# Autodesk Inventor assembly: Rack and Pinion Gearbox Assembly
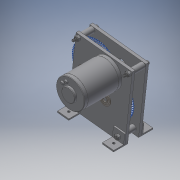
[picture p0: Inventor's stored thumbnail of the model, 180x180]
Saved by Autodesk Inventor 2018 (Build 220112000, 112)
## iProperties
Created: 2019-01-29
Part Number: Rack and Pinion Gearbox Assembly
Document SubType Name: Assembly
Designer: maste
Author: maste
## Documents named in this file (14)
- C:\Users\maste\OneDrive\Documents\GitHub\2019CAD\Drivebase but Calvin is a mad man\Rack and Pinion Gearbox Assembly.iam
- C:\Users\maste\OneDrive\Documents\GitHub\2019CAD\Drivebase but Calvin is a mad man\Rack and Pinion Gearbox Plate.ipt
- C:\Users\maste\OneDrive\Documents\GitHub\2019CAD\Drivebase but Calvin is a mad man\12t_Steel_Spur_Gear_20_DP_CIM_Motor_217-3099.ipt
- C:\Users\maste\OneDrive\Documents\GitHub\2019CAD\Drivebase but Calvin is a mad man\14t_Steel_Spur_Gear_20_DP_3_8_Hex_Bore_217-3100.step.ipt
- C:\Users\maste\OneDrive\Documents\GitHub\2019CAD\Drivebase but Calvin is a mad man\72t_Aluminum_Spur_Gear_20_DP_1_2_Hex_Bore_217-3576.ipt
- C:\Users\maste\OneDrive\Documents\GitHub\2019CAD\Drivebase but Calvin is a mad man\am-3832 375H to 500H Adapter.ipt
- C:\Users\maste\OneDrive\Documents\GitHub\2019CAD\Drivebase but Calvin is a mad man\Mini_CIM_Motor_217-3371.ipt
- C:\Users\maste\OneDrive\Documents\GitHub\2019CAD\Drivebase but Calvin is a mad man\10_25mm_3_8_ThunderHex_ID_x_0_875_OD_x_0_280_WD_Flanged_Bearing_217-5829 (1).ipt
- C:\Users\maste\OneDrive\Documents\GitHub\2019CAD\Drivebase but Calvin is a mad man\92196A272_18-8 STAINLESS STEEL SOCKET HEAD CAP SCREW.ipt
- C:\Users\maste\OneDrive\Documents\GitHub\2019CAD\Drivebase but Calvin is a mad man\Not Tiberculosis TB Hex Shaft.ipt
- C:\Users\maste\OneDrive\Documents\GitHub\2019CAD\Drivebase but Calvin is a mad man\I'm not awake enough to be making churros.ipt
- C:\Users\maste\OneDrive\Documents\GitHub\2019CAD\Drivebase but Calvin is a mad man\L-Bracket L.ipt
- C:\Users\maste\OneDrive\Documents\GitHub\2019CAD\Drivebase but Calvin is a mad man\92196A253_18-8 STAINLESS STEEL SOCKET HEAD CAP SCREW.ipt
- C:\Users\maste\OneDrive\Documents\GitHub\2019CAD\Drivebase but Calvin is a mad man\91831A011_TYPE 18-8 STAINLESS STL NYLON-INSERT LOCKNUT.ipt
## Components (33 placed, 13 different names)
1. Rack and Pinion Gearbox Plate:1 — Mate:79, Mate:80, Mate:81, Mate:82, Mate:94, Mate:95, Mate:97, Mate:98, Mate:99, Flush:4, Mate:101, Mate:102, Mate:103, Mate:105, Mate:106, Mate:107, Flush:5, Mate:109, Flush:6, Flush:7
2. Rack and Pinion Gearbox Plate:2 — Mate:68, Mate:69, Mate:70, Mate:71, Mate:72, Mate:73, Mate:74, Mate:75, Mate:76, Mate:77, Mate:78, Flush:6, Flush:7, Mate:110, Mate:111, Mate:112, Mate:113, Flush:8, Flush:9, Flush:10, Flush:11, Mate:114, Rotation:2, Rotation:3
3. 12t_Steel_Spur_Gear_20_DP_CIM_Motor_217-3099:1 — Mate:85, Flush:2, Mate:86
4. 14t_Steel_Spur_Gear_20_DP_3_8_Hex_Bore_217-3100.step:1 — Mate:21, Mate:22, Mate:92, Mate:93
5. 72t_Aluminum_Spur_Gear_20_DP_1_2_Hex_Bore_217-3576:1 — Mate:90, Mate:91, Flush:3
6. 72t_Aluminum_Spur_Gear_20_DP_1_2_Hex_Bore_217-3576:2 — Mate:83, Mate:84, Flush:1, Mate:89
7. am-3832 375H to 500H Adapter:1 — Mate:18, Mate:19, Mate:90, Mate:91, Flush:3, Mate:93
8. am-3832 375H to 500H Adapter:2 — Mate:32, Mate:33, Mate:83, Mate:84, Flush:1, Mate:87, Mate:88
9. Mini_CIM_Motor_217-3371:1 — Mate:68, Mate:69, Mate:70, Mate:85, Flush:2, Mate:86
10. 10_25mm_3_8_ThunderHex_ID_x_0_875_OD_x_0_280_WD_Flanged_Bearing_217-5829 (1):1 — Mate:73, Mate:74, Rotation:3
11. 10_25mm_3_8_ThunderHex_ID_x_0_875_OD_x_0_280_WD_Flanged_Bearing_217-5829 (1):2 — Mate:71, Mate:72, Rotation:1, Rotation:2
12. 10_25mm_3_8_ThunderHex_ID_x_0_875_OD_x_0_280_WD_Flanged_Bearing_217-5829 (1):3 — Mate:28, Mate:29, Mate:81, Mate:82, Mate:89
13. 10_25mm_3_8_ThunderHex_ID_x_0_875_OD_x_0_280_WD_Flanged_Bearing_217-5829 (1):4 — Mate:16, Mate:17, Mate:79, Mate:80, Mate:92
14. 92196A272_18-8 STAINLESS STEEL SOCKET HEAD CAP SCREW:1 — Mate:75, Mate:76
15. 92196A272_18-8 STAINLESS STEEL SOCKET HEAD CAP SCREW:2 — Mate:77, Mate:78
16. Not Tiberculosis TB Hex Shaft:1 — Mate:16, Mate:17, Mate:18, Mate:19, Mate:21, Mate:22, Rotation:1
17. Not Tiberculosis TB Hex Shaft:2 — Mate:28, Mate:29, Mate:32, Mate:33, Mate:87, Mate:88
18. I'm not awake enough to be making churros:1 — Mate:104, Mate:105
19. I'm not awake enough to be making churros:2 — Mate:96, Mate:97, Mate:110
20. I'm not awake enough to be making churros:3 — Mate:100, Mate:101
21. I'm not awake enough to be making churros:4 — Mate:108, Mate:109
22. L-Bracket L:1 — Mate:55, Mate:58, Mate:99, Flush:4
23. L-Bracket L:2 — Mate:54, Mate:59, Mate:107, Flush:5
24. L-Bracket L:3 — Mate:63, Flush:10, Flush:11, Mate:114
25. L-Bracket L:4 — Mate:62, Mate:113, Flush:8, Flush:9
26. 92196A253_18-8 STAINLESS STEEL SOCKET HEAD CAP SCREW:1 — Mate:54, Mate:59, Mate:65, Mate:106, Mate:108
27. 92196A253_18-8 STAINLESS STEEL SOCKET HEAD CAP SCREW:2 — Mate:55, Mate:58, Mate:64, Mate:98, Mate:100
28. 92196A253_18-8 STAINLESS STEEL SOCKET HEAD CAP SCREW:3 — Mate:67, Mate:94, Mate:95, Mate:96
29. 92196A253_18-8 STAINLESS STEEL SOCKET HEAD CAP SCREW:4 — Mate:66, Mate:102, Mate:103, Mate:104
30. 91831A011_TYPE 18-8 STAINLESS STL NYLON-INSERT LOCKNUT:1 — Mate:62, Mate:64
31. 91831A011_TYPE 18-8 STAINLESS STL NYLON-INSERT LOCKNUT:2 — Mate:63, Mate:65
32. 91831A011_TYPE 18-8 STAINLESS STL NYLON-INSERT LOCKNUT:3 — Mate:67, Mate:111
33. 91831A011_TYPE 18-8 STAINLESS STL NYLON-INSERT LOCKNUT:4 — Mate:66, Mate:112
## Relationships (81: Mate 67, Flush 11, RelateRotation 3)
- Mate:16: 10_25mm_3_8_ThunderHex_ID_x_0_875_OD_x_0_280_WD_Flanged_Bearing_217-5829 (1):4 ↔ Not Tiberculosis TB Hex Shaft:1
- Mate:17: 10_25mm_3_8_ThunderHex_ID_x_0_875_OD_x_0_280_WD_Flanged_Bearing_217-5829 (1):4 ↔ Not Tiberculosis TB Hex Shaft:1
- Mate:18: am-3832 375H to 500H Adapter:1 ↔ Not Tiberculosis TB Hex Shaft:1
- Mate:19: am-3832 375H to 500H Adapter:1 ↔ Not Tiberculosis TB Hex Shaft:1
- Mate:21: 14t_Steel_Spur_Gear_20_DP_3_8_Hex_Bore_217-3100.step:1 ↔ Not Tiberculosis TB Hex Shaft:1
- Mate:22: 14t_Steel_Spur_Gear_20_DP_3_8_Hex_Bore_217-3100.step:1 ↔ Not Tiberculosis TB Hex Shaft:1
- Mate:28: 10_25mm_3_8_ThunderHex_ID_x_0_875_OD_x_0_280_WD_Flanged_Bearing_217-5829 (1):3 ↔ Not Tiberculosis TB Hex Shaft:2
- Mate:29: 10_25mm_3_8_ThunderHex_ID_x_0_875_OD_x_0_280_WD_Flanged_Bearing_217-5829 (1):3 ↔ Not Tiberculosis TB Hex Shaft:2
- Mate:32: am-3832 375H to 500H Adapter:2 ↔ Not Tiberculosis TB Hex Shaft:2
- Mate:33: am-3832 375H to 500H Adapter:2 ↔ Not Tiberculosis TB Hex Shaft:2
- Mate:54: L-Bracket L:2 ↔ 92196A253_18-8 STAINLESS STEEL SOCKET HEAD CAP SCREW:1
- Mate:55: L-Bracket L:1 ↔ 92196A253_18-8 STAINLESS STEEL SOCKET HEAD CAP SCREW:2
- Mate:58: L-Bracket L:1 ↔ 92196A253_18-8 STAINLESS STEEL SOCKET HEAD CAP SCREW:2
- Mate:59: L-Bracket L:2 ↔ 92196A253_18-8 STAINLESS STEEL SOCKET HEAD CAP SCREW:1
- Mate:62: L-Bracket L:4 ↔ 91831A011_TYPE 18-8 STAINLESS STL NYLON-INSERT LOCKNUT:1
- Mate:63: L-Bracket L:3 ↔ 91831A011_TYPE 18-8 STAINLESS STL NYLON-INSERT LOCKNUT:2
- Mate:64: 92196A253_18-8 STAINLESS STEEL SOCKET HEAD CAP SCREW:2 ↔ 91831A011_TYPE 18-8 STAINLESS STL NYLON-INSERT LOCKNUT:1
- Mate:65: 92196A253_18-8 STAINLESS STEEL SOCKET HEAD CAP SCREW:1 ↔ 91831A011_TYPE 18-8 STAINLESS STL NYLON-INSERT LOCKNUT:2
- Mate:66: 92196A253_18-8 STAINLESS STEEL SOCKET HEAD CAP SCREW:4 ↔ 91831A011_TYPE 18-8 STAINLESS STL NYLON-INSERT LOCKNUT:4
- Mate:67: 92196A253_18-8 STAINLESS STEEL SOCKET HEAD CAP SCREW:3 ↔ 91831A011_TYPE 18-8 STAINLESS STL NYLON-INSERT LOCKNUT:3
- Mate:68: Rack and Pinion Gearbox Plate:2 ↔ Mini_CIM_Motor_217-3371:1
- Mate:69: Rack and Pinion Gearbox Plate:2 ↔ Mini_CIM_Motor_217-3371:1
- Mate:70: Rack and Pinion Gearbox Plate:2 ↔ Mini_CIM_Motor_217-3371:1
- Mate:71: Rack and Pinion Gearbox Plate:2 ↔ 10_25mm_3_8_ThunderHex_ID_x_0_875_OD_x_0_280_WD_Flanged_Bearing_217-5829 (1):2
- Mate:72: Rack and Pinion Gearbox Plate:2 ↔ 10_25mm_3_8_ThunderHex_ID_x_0_875_OD_x_0_280_WD_Flanged_Bearing_217-5829 (1):2
- Mate:73: Rack and Pinion Gearbox Plate:2 ↔ 10_25mm_3_8_ThunderHex_ID_x_0_875_OD_x_0_280_WD_Flanged_Bearing_217-5829 (1):1
- Mate:74: Rack and Pinion Gearbox Plate:2 ↔ 10_25mm_3_8_ThunderHex_ID_x_0_875_OD_x_0_280_WD_Flanged_Bearing_217-5829 (1):1
- Mate:75: Rack and Pinion Gearbox Plate:2 ↔ 92196A272_18-8 STAINLESS STEEL SOCKET HEAD CAP SCREW:1
- Mate:76: Rack and Pinion Gearbox Plate:2 ↔ 92196A272_18-8 STAINLESS STEEL SOCKET HEAD CAP SCREW:1
- Mate:77: Rack and Pinion Gearbox Plate:2 ↔ 92196A272_18-8 STAINLESS STEEL SOCKET HEAD CAP SCREW:2
- Mate:78: Rack and Pinion Gearbox Plate:2 ↔ 92196A272_18-8 STAINLESS STEEL SOCKET HEAD CAP SCREW:2
- Mate:79: Rack and Pinion Gearbox Plate:1 ↔ 10_25mm_3_8_ThunderHex_ID_x_0_875_OD_x_0_280_WD_Flanged_Bearing_217-5829 (1):4
- Mate:80: Rack and Pinion Gearbox Plate:1 ↔ 10_25mm_3_8_ThunderHex_ID_x_0_875_OD_x_0_280_WD_Flanged_Bearing_217-5829 (1):4
- Mate:81: Rack and Pinion Gearbox Plate:1 ↔ 10_25mm_3_8_ThunderHex_ID_x_0_875_OD_x_0_280_WD_Flanged_Bearing_217-5829 (1):3
- Mate:82: Rack and Pinion Gearbox Plate:1 ↔ 10_25mm_3_8_ThunderHex_ID_x_0_875_OD_x_0_280_WD_Flanged_Bearing_217-5829 (1):3
- Mate:83: 72t_Aluminum_Spur_Gear_20_DP_1_2_Hex_Bore_217-3576:2 ↔ am-3832 375H to 500H Adapter:2
- Mate:84: 72t_Aluminum_Spur_Gear_20_DP_1_2_Hex_Bore_217-3576:2 ↔ am-3832 375H to 500H Adapter:2
- Flush:1: 72t_Aluminum_Spur_Gear_20_DP_1_2_Hex_Bore_217-3576:2 ↔ am-3832 375H to 500H Adapter:2
- Mate:85: 12t_Steel_Spur_Gear_20_DP_CIM_Motor_217-3099:1 ↔ Mini_CIM_Motor_217-3371:1
- Flush:2: 12t_Steel_Spur_Gear_20_DP_CIM_Motor_217-3099:1 ↔ Mini_CIM_Motor_217-3371:1
- Mate:86: 12t_Steel_Spur_Gear_20_DP_CIM_Motor_217-3099:1 ↔ Mini_CIM_Motor_217-3371:1
- Mate:87: am-3832 375H to 500H Adapter:2 ↔ Not Tiberculosis TB Hex Shaft:2
- Mate:88: am-3832 375H to 500H Adapter:2 ↔ Not Tiberculosis TB Hex Shaft:2
- Mate:89: 72t_Aluminum_Spur_Gear_20_DP_1_2_Hex_Bore_217-3576:2 ↔ 10_25mm_3_8_ThunderHex_ID_x_0_875_OD_x_0_280_WD_Flanged_Bearing_217-5829 (1):3
- Mate:90: 72t_Aluminum_Spur_Gear_20_DP_1_2_Hex_Bore_217-3576:1 ↔ am-3832 375H to 500H Adapter:1
- Mate:91: 72t_Aluminum_Spur_Gear_20_DP_1_2_Hex_Bore_217-3576:1 ↔ am-3832 375H to 500H Adapter:1
- Flush:3: 72t_Aluminum_Spur_Gear_20_DP_1_2_Hex_Bore_217-3576:1 ↔ am-3832 375H to 500H Adapter:1
- Mate:92: 14t_Steel_Spur_Gear_20_DP_3_8_Hex_Bore_217-3100.step:1 ↔ 10_25mm_3_8_ThunderHex_ID_x_0_875_OD_x_0_280_WD_Flanged_Bearing_217-5829 (1):4
- Mate:93: 14t_Steel_Spur_Gear_20_DP_3_8_Hex_Bore_217-3100.step:1 ↔ am-3832 375H to 500H Adapter:1
- Mate:94: Rack and Pinion Gearbox Plate:1 ↔ 92196A253_18-8 STAINLESS STEEL SOCKET HEAD CAP SCREW:3
- Mate:95: Rack and Pinion Gearbox Plate:1 ↔ 92196A253_18-8 STAINLESS STEEL SOCKET HEAD CAP SCREW:3
- Mate:96: I'm not awake enough to be making churros:2 ↔ 92196A253_18-8 STAINLESS STEEL SOCKET HEAD CAP SCREW:3
- Mate:97: Rack and Pinion Gearbox Plate:1 ↔ I'm not awake enough to be making churros:2
- Mate:98: Rack and Pinion Gearbox Plate:1 ↔ 92196A253_18-8 STAINLESS STEEL SOCKET HEAD CAP SCREW:2
- Mate:99: Rack and Pinion Gearbox Plate:1 ↔ L-Bracket L:1
- Flush:4: Rack and Pinion Gearbox Plate:1 ↔ L-Bracket L:1
- Mate:100: I'm not awake enough to be making churros:3 ↔ 92196A253_18-8 STAINLESS STEEL SOCKET HEAD CAP SCREW:2
- Mate:101: Rack and Pinion Gearbox Plate:1 ↔ I'm not awake enough to be making churros:3
- Mate:102: Rack and Pinion Gearbox Plate:1 ↔ 92196A253_18-8 STAINLESS STEEL SOCKET HEAD CAP SCREW:4
- Mate:103: Rack and Pinion Gearbox Plate:1 ↔ 92196A253_18-8 STAINLESS STEEL SOCKET HEAD CAP SCREW:4
- Mate:104: I'm not awake enough to be making churros:1 ↔ 92196A253_18-8 STAINLESS STEEL SOCKET HEAD CAP SCREW:4
- Mate:105: Rack and Pinion Gearbox Plate:1 ↔ I'm not awake enough to be making churros:1
- Mate:106: Rack and Pinion Gearbox Plate:1 ↔ 92196A253_18-8 STAINLESS STEEL SOCKET HEAD CAP SCREW:1
- Mate:107: Rack and Pinion Gearbox Plate:1 ↔ L-Bracket L:2
- Flush:5: Rack and Pinion Gearbox Plate:1 ↔ L-Bracket L:2
- Mate:108: I'm not awake enough to be making churros:4 ↔ 92196A253_18-8 STAINLESS STEEL SOCKET HEAD CAP SCREW:1
- Mate:109: Rack and Pinion Gearbox Plate:1 ↔ I'm not awake enough to be making churros:4
- Flush:6: Rack and Pinion Gearbox Plate:1 ↔ Rack and Pinion Gearbox Plate:2
- Flush:7: Rack and Pinion Gearbox Plate:1 ↔ Rack and Pinion Gearbox Plate:2
- Mate:110: Rack and Pinion Gearbox Plate:2 ↔ I'm not awake enough to be making churros:2
- Mate:111: Rack and Pinion Gearbox Plate:2 ↔ 91831A011_TYPE 18-8 STAINLESS STL NYLON-INSERT LOCKNUT:3
- Mate:112: Rack and Pinion Gearbox Plate:2 ↔ 91831A011_TYPE 18-8 STAINLESS STL NYLON-INSERT LOCKNUT:4
- Mate:113: Rack and Pinion Gearbox Plate:2 ↔ L-Bracket L:4
- Flush:8: Rack and Pinion Gearbox Plate:2 ↔ L-Bracket L:4
- Flush:9: Rack and Pinion Gearbox Plate:2 ↔ L-Bracket L:4
- Flush:10: Rack and Pinion Gearbox Plate:2 ↔ L-Bracket L:3
- Flush:11: Rack and Pinion Gearbox Plate:2 ↔ L-Bracket L:3
- Mate:114: Rack and Pinion Gearbox Plate:2 ↔ L-Bracket L:3
- Rotation:1 [RelateRotation] (1 ul): 10_25mm_3_8_ThunderHex_ID_x_0_875_OD_x_0_280_WD_Flanged_Bearing_217-5829 (1):2 ↔ Not Tiberculosis TB Hex Shaft:1
- Rotation:2 [RelateRotation] (1 ul): Rack and Pinion Gearbox Plate:2 ↔ 10_25mm_3_8_ThunderHex_ID_x_0_875_OD_x_0_280_WD_Flanged_Bearing_217-5829 (1):2
- Rotation:3 [RelateRotation] (1 ul): Rack and Pinion Gearbox Plate:2 ↔ 10_25mm_3_8_ThunderHex_ID_x_0_875_OD_x_0_280_WD_Flanged_Bearing_217-5829 (1):1
